# Autodesk Inventor assembly: Assembly of Sorting
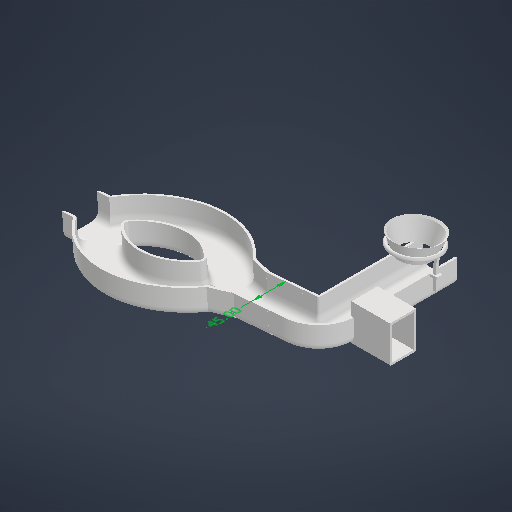
[picture p0: Inventor's stored thumbnail of the model, 512x512]
Saved by Autodesk Inventor 2026.2 (Build 302298010, 298A)
## iProperties
Created: 2026-04-15
Part Number: Assembly of Sorting
Document SubType Name: Assembly
Designer: lenovo
Author: lenovo
## Documents named in this file (6)
- F:\Semester 4\Basics of Mechatronics\Project\Assembly of Sorting .iam
- F:\Semester 4\Basics of Mechatronics\Project\path.ipt
- F:\Semester 4\Basics of Mechatronics\Project\Base of Sorting.ipt
- F:\Semester 4\Basics of Mechatronics\Project\Path from IR to PIN.ipt
- F:\Semester 4\Basics of Mechatronics\Project\Basket Holder 2 .ipt
- F:\Semester 4\Basics of Mechatronics\Project\basket.ipt
## Components (5 placed, 5 different names)
1. Path:1 — Mate:8, Mate:9, Mate:10, Mate:18, Mate:19, Mate:20, Mate:21, Mate:22
2. Path from IR to PIN:1 — Mate:8, Mate:9, Mate:10, Mate:11, Mate:12, Mate:13, Mate:18
3. Base of Sorting:1 — Mate:11, Mate:12, Mate:13
4. Basket Holder:1 — Mate:19, Mate:20, Mate:21, Mate:22, Mate:23
5. basket:1 — Mate:23
## Relationships (12: Mate 12)
- Mate:8: Path:1 ↔ Path from IR to PIN:1
- Mate:9: Path:1 ↔ Path from IR to PIN:1
- Mate:10: Path:1 ↔ Path from IR to PIN:1
- Mate:11: Path from IR to PIN:1 ↔ Base of Sorting:1
- Mate:12: Path from IR to PIN:1 ↔ Base of Sorting:1
- Mate:13: Path from IR to PIN:1 ↔ Base of Sorting:1
- Mate:18: Path:1 ↔ Path from IR to PIN:1
- Mate:19: Path:1 ↔ Basket Holder:1
- Mate:20: Path:1 ↔ Basket Holder:1
- Mate:21: Path:1 ↔ Basket Holder:1
- Mate:22: Path:1 ↔ Basket Holder:1
- Mate:23: Basket Holder:1 ↔ basket:1
